# Autodesk Inventor assembly: frame
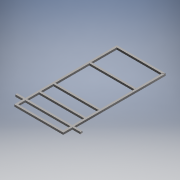
[picture p0: Inventor's stored thumbnail of the model, 180x180]
Saved by Autodesk Inventor 2019 (Build 230136000, 136)
## iProperties
Created: 2019-04-23
Part Number: frame
Document SubType Name: Weldment
Designer: Callum Snowden
Weld Material: Welded Aluminum-6061
Mass: 16255.4 g
Surface Area: 16616.8 cm^2
Volume: 2070.75 cm^3
Density: 7.85 g/cm^3
Author: Callum Snowden
## Documents named in this file (13)
- C:\Users\callum.snowden\Documents\GitHub\clasohlsonkart\mechanical\frame\frame.iam
- C:\Users\callum.snowden\Documents\GitHub\clasohlsonkart\mechanical\frame\750mm_box_section.ipt
- C:\Users\callum.snowden\Documents\GitHub\clasohlsonkart\mechanical\frame\1500mm_box_section.ipt
- C:\Users\callum.snowden\Documents\GitHub\clasohlsonkart\mechanical\frame\1500mm_box_section_MIR.ipt
- C:\Users\callum.snowden\Documents\GitHub\clasohlsonkart\mechanical\frame\690mm_box_section.ipt
- C:\Users\callum.snowden\Documents\GitHub\clasohlsonkart\mechanical\frame\1250mm_box_section.ipt
- C:\Users\callum.snowden\Documents\GitHub\clasohlsonkart\mechanical\frame\140mm_box_section.ipt
- C:\Users\callum.snowden\Documents\GitHub\clasohlsonkart\mechanical\frame\frame\AIP\FEA\cutzhkwf4.fins
- C:\Users\callum.snowden\Documents\GitHub\clasohlsonkart\mechanical\frame\frame\AIP\FEA\cutzhkwg0.fsat
- C:\Users\callum.snowden\Documents\GitHub\clasohlsonkart\mechanical\frame\frame\AIP\FEA\cutzhkwg0.ftes
- C:\Users\callum.snowden\Documents\GitHub\clasohlsonkart\mechanical\frame\frame\AIP\FEA\cutzhkwg0.fwiz
- C:\Users\callum.snowden\Documents\GitHub\clasohlsonkart\mechanical\frame\frame\AIP\FEA\cutzhkwio.fmsh
- C:\Users\callum.snowden\Documents\GitHub\clasohlsonkart\mechanical\frame\frame\AIP\FEA\cutzhkwip.fres
## Components (10 placed, 6 different names)
1. 750mm_box_section:1 — Rigid:11
2. 750mm_box_section:2 — Rigid:3, Rigid:8
3. 1500mm_box_section:1 — Rigid:3, Rigid:4, Rigid:5, Rigid:6
4. 1500mm_box_section_MIR:1 — Rigid:7, Rigid:8
5. 690mm_box_section:1 — Rigid:4
6. 690mm_box_section:2 — Rigid:6
7. 690mm_box_section:3 — Rigid:5
8. 1250mm_box_section:1 — Rigid:7, Rigid:9, Rigid:10
9. 140mm_box_section:1 — Rigid:10
10. 140mm_box_section:2 — Rigid:9, Rigid:11
## Relationships (9: WeldJoint 9)
- Rigid:3 [WeldJoint]: 750mm_box_section:2 ↔ 1500mm_box_section:1
- Rigid:4 [WeldJoint]: 1500mm_box_section:1 ↔ 690mm_box_section:1
- Rigid:5 [WeldJoint]: 1500mm_box_section:1 ↔ 690mm_box_section:3
- Rigid:6 [WeldJoint]: 1500mm_box_section:1 ↔ 690mm_box_section:2
- Rigid:7 [WeldJoint]: 1500mm_box_section_MIR:1 ↔ 1250mm_box_section:1
- Rigid:8 [WeldJoint]: 750mm_box_section:2 ↔ 1500mm_box_section_MIR:1
- Rigid:9 [WeldJoint]: 1250mm_box_section:1 ↔ 140mm_box_section:2
- Rigid:10 [WeldJoint]: 1250mm_box_section:1 ↔ 140mm_box_section:1
- Rigid:11 [WeldJoint]: 750mm_box_section:1 ↔ 140mm_box_section:2
## Named parameters: sa_0 = 0, sa_1 = 0, sa_2 = -100000
note: some values were not read from the file. Shown as the stored number, unit unknown: "sa_0", "sa_1", "sa_2".
